# Autodesk Inventor assembly: lidarm
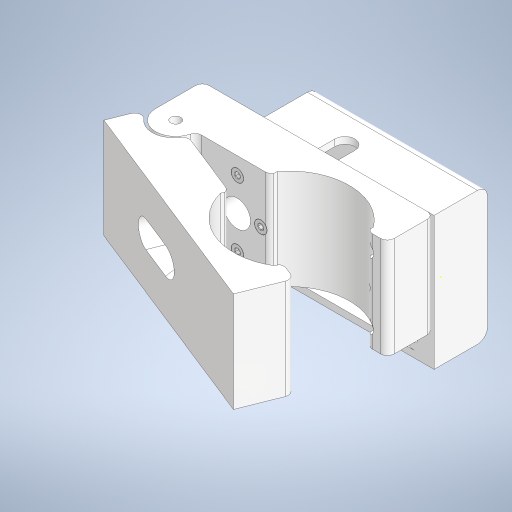
[picture p0: Inventor's stored thumbnail of the model, 512x512]
Saved by Autodesk Inventor 2023.1 (Build 271208000, 208)
## iProperties
Created: 2023-03-22
Part Number: lidarm
Document SubType Name: Assembly
Designer: liaar
Author: liaar
## Documents named in this file (7)
- C:\Users\liaar\OneDrive\Desktop\Capstone\lidarm.iam
- C:\Users\liaar\OneDrive\Desktop\Capstone\lidarhouse.ipt
- C:\Users\liaar\OneDrive\Desktop\Capstone\Bike_Mount_Right_v2.ipt
- C:\Users\liaar\OneDrive\Desktop\Capstone\lidarsensor.ipt
- C:\Users\liaar\Downloads\BOLT.ipt
- C:\Users\liaar\Downloads\NUT.ipt
- C:\Users\liaar\Downloads\Bike_Mount_Left.ipt
## Components (16 placed, 6 different names)
1. lidarhouse:1 — Flush:1, Flush:2, Flush:3, Mate:1, Mate:2, Flush:6, Flush:7, Flush:8, Flush:12, Flush:13, Flush:14, Flush:15
2. Bike_Mount_Right_v2:1 — Mate:2, Flush:6, Flush:7, Mate:3, Flush:9, Mate:4, Mate:5, Mate:6, Mate:7, Mate:8, Flush:10, Flush:11, Mate:9, Mate:10, Mate:11, Mate:18, Mate:19, Flush:16
3. lidarsensor:1 — Mate:1, Flush:8, Mate:18
4. BOLT:1 — Mate:7, Mate:10, Mate:16
5. BOLT:2 — Mate:3, Flush:9, Mate:14
6. BOLT:3 — Mate:8, Mate:9, Mate:12
7. BOLT:4 — Mate:6, Mate:11, Mate:15
8. BOLT:5 — Mate:5, Flush:11, Mate:13
9. BOLT:6 — Mate:4, Flush:10, Mate:17
10. NUT:1 — Mate:13, Flush:13
11. NUT:2 — Mate:15, Flush:15
12. NUT:3 — Mate:12, Flush:12
13. NUT:4 — Mate:14, Flush:14
14. NUT:5 — Mate:16
15. NUT:6 — Mate:17
16. Bike_Mount_Left:1 — Mate:19, Flush:16
## Relationships (33: Mate 19, Flush 14)
- Flush:1: lidarhouse:1
- Flush:2: lidarhouse:1
- Flush:3: lidarhouse:1
- Mate:1 (4 mm): lidarhouse:1 ↔ lidarsensor:1
- Mate:2: lidarhouse:1 ↔ Bike_Mount_Right_v2:1
- Flush:6: lidarhouse:1 ↔ Bike_Mount_Right_v2:1
- Flush:7: lidarhouse:1 ↔ Bike_Mount_Right_v2:1
- Flush:8 (1.75 mm): lidarhouse:1 ↔ lidarsensor:1
- Mate:3: Bike_Mount_Right_v2:1 ↔ BOLT:2
- Flush:9: Bike_Mount_Right_v2:1 ↔ BOLT:2
- Mate:4: Bike_Mount_Right_v2:1 ↔ BOLT:6
- Mate:5: Bike_Mount_Right_v2:1 ↔ BOLT:5
- Mate:6: Bike_Mount_Right_v2:1 ↔ BOLT:4
- Mate:7: Bike_Mount_Right_v2:1 ↔ BOLT:1
- Mate:8: Bike_Mount_Right_v2:1 ↔ BOLT:3
- Flush:10: Bike_Mount_Right_v2:1 ↔ BOLT:6
- Flush:11: Bike_Mount_Right_v2:1 ↔ BOLT:5
- Mate:9: Bike_Mount_Right_v2:1 ↔ BOLT:3
- Mate:10: Bike_Mount_Right_v2:1 ↔ BOLT:1
- Mate:11: Bike_Mount_Right_v2:1 ↔ BOLT:4
- Mate:12: BOLT:3 ↔ NUT:3
- Flush:12: lidarhouse:1 ↔ NUT:3
- Mate:13: BOLT:5 ↔ NUT:1
- Flush:13: lidarhouse:1 ↔ NUT:1
- Mate:14: BOLT:2 ↔ NUT:4
- Flush:14: lidarhouse:1 ↔ NUT:4
- Mate:15: BOLT:4 ↔ NUT:2
- Flush:15: lidarhouse:1 ↔ NUT:2
- Mate:16: BOLT:1 ↔ NUT:5
- Mate:17: BOLT:6 ↔ NUT:6
- Mate:18: Bike_Mount_Right_v2:1 ↔ lidarsensor:1
- Mate:19: Bike_Mount_Right_v2:1 ↔ Bike_Mount_Left:1
- Flush:16: Bike_Mount_Right_v2:1 ↔ Bike_Mount_Left:1
